# Autodesk Inventor assembly: Lever
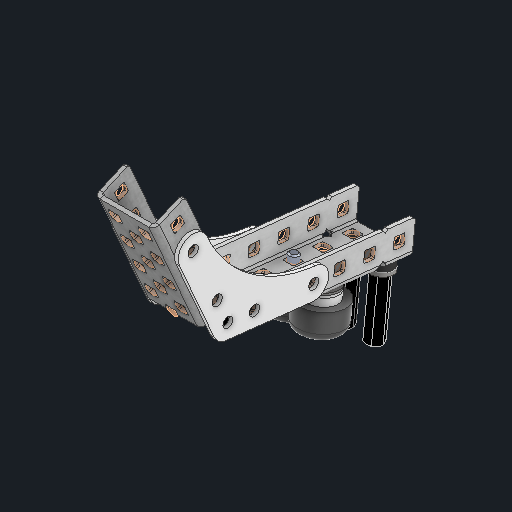
[picture p0: Inventor's stored thumbnail of the model, 512x512]
Saved by Autodesk Inventor 2025 (Build 290162000, 162)
## iProperties
Created: 2024-10-22
Part Number: Lever
Document SubType Name: Assembly
Designer: averey
Author: averey
## Documents named in this file (17)
- D:\VEX\High Stakes\CAD\V2\Clamp\Lever.iam
- D:\VEX\High Stakes\CAD\ROBOPROS-CAD-Inventor\Structure\C Channel\Aluminum 1x2x1\Alu C 1x2x1x5.ipt
- D:\VEX\High Stakes\CAD\V2\Clamp\Custom Parts\60 Degree Gusset.ipt
- D:\VEX\High Stakes\CAD\ROBOPROS-CAD-Inventor\Structure\Standoff\Standoff 1.00.ipt
- D:\VEX\High Stakes\CAD\ROBOPROS-CAD-Inventor\Structure\C Channel\Aluminum 1x2x1\Alu C 1x2x1x4.ipt
- D:\VEX\High Stakes\CAD\ROBOPROS-CAD-Inventor\Structure\C Channel\Aluminum 1x2x1\Alu C 1x2x1x6.ipt
- D:\VEX\High Stakes\CAD\ROBOPROS-CAD-Inventor\Motion\Spacers\Spacer Nylon .375 OD.ipt
- D:\VEX\High Stakes\CAD\ROBOPROS-CAD-Inventor\Structure\Hardware\Rubber Bumper Smooth.ipt
- D:\VEX\High Stakes\CAD\ROBOPROS-CAD-Inventor\Structure\Standoff.ipt
- D:\VEX\High Stakes\CAD\ROBOPROS-CAD-Inventor\Motion\Spacers\Washer Steel\SWasher .375 OD x .062500.ipt
- D:\VEX\High Stakes\CAD\ROBOPROS-CAD-Inventor\Motion\Spacers\Washer Steel.ipt
- D:\VEX\High Stakes\CAD\ROBOPROS-CAD-Inventor\Motion\Spacers\Spacer Nylon .375 OD\NSpacer .375 OD x .125.ipt
- D:\VEX\High Stakes\CAD\ROBOPROS-CAD-Inventor\Motion\Spacers\Spacer Nylon .500 OD\NSpacer White .500 OD x .125.ipt
- D:\VEX\High Stakes\CAD\ROBOPROS-CAD-Inventor\Motion\Spacers\Spacer Nylon .500 OD.ipt
- D:\VEX\High Stakes\CAD\ROBOPROS-CAD-Inventor\Motion\Spacers\Washer Teflon\TWasher .500 OD x .04000.ipt
- D:\VEX\High Stakes\CAD\ROBOPROS-CAD-Inventor\Motion\Spacers\Washer Teflon.ipt
- D:\VEX\High Stakes\CAD\ROBOPROS-CAD-Inventor\Motion\Spacers\Washer Steel\SWasher .500 OD x .031250.ipt
## Components (20 placed, 11 different names)
1. Alu C 1x2x1x5:2 — Insert:2, Mate:1, Insert:3, Mate:3, Insert:6, Mate:7
2. 60 Degree Gusset:1 — Insert:2, Mate:1, Mate:5, Insert:5, Mate:6
3. 60 Degree Gusset:2 — Insert:3, Mate:3, Insert:4
4. Standoff 1.00:1 — Insert:4, Mate:5
5. Alu C 1x2x1x4:1 — Insert:5, Mate:6
6. Alu C 1x2x1x6:1 — Insert:6, Mate:7, Insert:7, Insert:12, Insert:19, Insert:20
7. Standoff 1.00:2 — Insert:9
8. SWasher .375 OD x .062500:1 — Insert:8, Insert:9
9. NSpacer .375 OD x .125:1 — Insert:7, Insert:8
10. Standoff 1.00:3
11. SWasher .375 OD x .062500:2
12. NSpacer .375 OD x .125:2 — Insert:12
13. Rubber Bumper Smooth:1 — Insert:15
14. NSpacer White .500 OD x .125:1 — Insert:14, Insert:15
15. TWasher .500 OD x .04000:1 — Insert:13, Insert:14
16. SWasher .500 OD x .031250:3 — Insert:13, Insert:20
17. Rubber Bumper Smooth:2
18. NSpacer White .500 OD x .125:2
19. TWasher .500 OD x .04000:2
20. SWasher .500 OD x .031250:4 — Insert:19
## Relationships (24: Insert 19, Mate 5)
- Insert:2: Alu C 1x2x1x5:2 ↔ 60 Degree Gusset:1
- Mate:1: Alu C 1x2x1x5:2 ↔ 60 Degree Gusset:1
- Insert:3: Alu C 1x2x1x5:2 ↔ 60 Degree Gusset:2
- Mate:3: Alu C 1x2x1x5:2 ↔ 60 Degree Gusset:2
- Insert:4: 60 Degree Gusset:2 ↔ Standoff 1.00:1
- Mate:5: 60 Degree Gusset:1 ↔ Standoff 1.00:1
- Insert:5: 60 Degree Gusset:1 ↔ Alu C 1x2x1x4:1
- Mate:6: 60 Degree Gusset:1 ↔ Alu C 1x2x1x4:1
- Insert:6: Alu C 1x2x1x5:2 ↔ Alu C 1x2x1x6:1
- Mate:7: Alu C 1x2x1x5:2 ↔ Alu C 1x2x1x6:1
- Insert:7: Alu C 1x2x1x6:1 ↔ NSpacer .375 OD x .125:1
- Insert:8: SWasher .375 OD x .062500:1 ↔ NSpacer .375 OD x .125:1
- Insert:9: Standoff 1.00:2 ↔ SWasher .375 OD x .062500:1
- [Insert]: SWasher .375 OD x .062500:2 ↔ NSpacer .375 OD x .125:2
- [Insert]: Standoff 1.00:3 ↔ SWasher .375 OD x .062500:2
- Insert:12: Alu C 1x2x1x6:1 ↔ NSpacer .375 OD x .125:2
- Insert:13: TWasher .500 OD x .04000:1 ↔ SWasher .500 OD x .031250:3
- Insert:14: NSpacer White .500 OD x .125:1 ↔ TWasher .500 OD x .04000:1
- Insert:15: Rubber Bumper Smooth:1 ↔ NSpacer White .500 OD x .125:1
- [Insert]: TWasher .500 OD x .04000:2 ↔ SWasher .500 OD x .031250:4
- [Insert]: NSpacer White .500 OD x .125:2 ↔ TWasher .500 OD x .04000:2
- [Insert]: Rubber Bumper Smooth:2 ↔ NSpacer White .500 OD x .125:2
- Insert:19: Alu C 1x2x1x6:1 ↔ SWasher .500 OD x .031250:4
- Insert:20: Alu C 1x2x1x6:1 ↔ SWasher .500 OD x .031250:3
## Named parameters: d38_d36 = 0 mm, d39_d37 = 0 mm, d44_d41 = 0 mm, d45_d42 = 0 mm, d46_d43 = 0 mm
